# Autodesk Inventor assembly: 000.200 - Основание
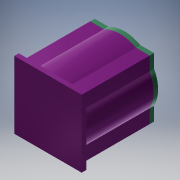
[picture p0: Inventor's stored thumbnail of the model, 180x180]
Saved by Autodesk Inventor 2019 (Build 230136000, 136)
## iProperties
Created: 2020-03-17
Part Number: 000.200 - Основание
Material: Типовые
Document SubType Name: Assembly
Designer: Петров Иван
Author: Петров Иван
## Documents named in this file (7)
- E:\IVAN\Ivan_desktop\GitHub\Manipulation_IRS\hardware\SCARA\000.200 - Основание.iam
- E:\IVAN\Ivan_desktop\GitHub\Manipulation_IRS\hardware\SCARA\000.201 - Станина.ipt
- E:\IVAN\Ivan_desktop\GitHub\Manipulation_IRS\hardware\SCARA\000.202 - Крышка.ipt
- E:\IVAN\Ivan_desktop\GitHub\Manipulation_IRS\hardware\SCARA\components\Подшипник 25х47х8 7000105.ipt
- E:\IVAN\Ivan_desktop\GitHub\Manipulation_IRS\hardware\SCARA\000.203 - База подшипника.ipt
- E:\IVAN\Ivan_desktop\GitHub\Manipulation_IRS\hardware\SCARA\components\Dynamixel MX-106.iam
- E:\IVAN\Ivan_desktop\GitHub\Manipulation_IRS\hardware\SCARA\000.204 - Поворотное основание.ipt
## Components (6 placed, 6 different names)
1. 000.201 - Станина:1 — Совмещение:8, Совмещение:9, Совмещение:16
2. 000.202 - Крышка:1 — Совмещение:8, Совмещение:9, Совмещение:16, Совмещение:17, Совмещение:18, Совмещение:19, Совмещение:22, Совмещение:23, Совмещение:24
3. Подшипник 25х47х8 7000105:1 — Совмещение:20, Совмещение:21, Совмещение:26
4. 000.203 - База подшипника:1 — Совмещение:17, Совмещение:18, Совмещение:19, Совмещение:20, Совмещение:21
5. Dynamixel MX-106:1 [sub-assembly] — Совмещение:22, Совмещение:23, Совмещение:24, Совмещение:25, Совмещение:27
6. 000.204 - Поворотное основание:1 — Совмещение:25, Совмещение:26, Совмещение:27
## Relationships (14: Mate 14)
- Совмещение:8 [Mate]: 000.201 - Станина:1 ↔ 000.202 - Крышка:1
- Совмещение:9 [Mate]: 000.201 - Станина:1 ↔ 000.202 - Крышка:1
- Совмещение:16 [Mate]: 000.201 - Станина:1 ↔ 000.202 - Крышка:1
- Совмещение:17 [Mate]: 000.202 - Крышка:1 ↔ 000.203 - База подшипника:1
- Совмещение:18 [Mate]: 000.202 - Крышка:1 ↔ 000.203 - База подшипника:1
- Совмещение:19 [Mate]: 000.202 - Крышка:1 ↔ 000.203 - База подшипника:1
- Совмещение:20 [Mate]: Подшипник 25х47х8 7000105:1 ↔ 000.203 - База подшипника:1
- Совмещение:21 [Mate]: Подшипник 25х47х8 7000105:1 ↔ 000.203 - База подшипника:1
- Совмещение:22 [Mate]: 000.202 - Крышка:1 ↔ Dynamixel MX-106:1
- Совмещение:23 [Mate]: 000.202 - Крышка:1 ↔ Dynamixel MX-106:1
- Совмещение:24 [Mate]: 000.202 - Крышка:1 ↔ Dynamixel MX-106:1
- Совмещение:25 [Mate]: Dynamixel MX-106:1 ↔ 000.204 - Поворотное основание:1
- Совмещение:26 [Mate]: Подшипник 25х47х8 7000105:1 ↔ 000.204 - Поворотное основание:1
- Совмещение:27 [Mate]: Dynamixel MX-106:1 ↔ 000.204 - Поворотное основание:1
